# Autodesk Inventor assembly: Lever
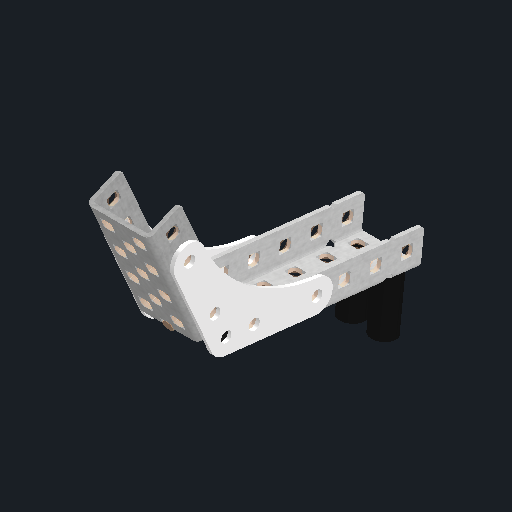
[picture p0: Inventor's stored thumbnail of the model, 512x512]
Saved by Autodesk Inventor 2025 (Build 290162000, 162)
## iProperties
Created: 2024-10-22
Part Number: Lever
Document SubType Name: Assembly
Designer: averey
Author: averey
## Documents named in this file (9)
- D:\VEX\High Stakes\CAD\V2\Clamp\Lever.iam
- D:\VEX\High Stakes\CAD\ROBOPROS-CAD-Inventor\Structure\C Channel\Aluminum 1x2x1\Alu C 1x2x1x5.ipt
- D:\VEX\High Stakes\CAD\V2\Clamp\Custom Parts\60 Degree Gusset.ipt
- D:\VEX\High Stakes\CAD\ROBOPROS-CAD-Inventor\Structure\Standoff\Standoff 1.00.ipt
- C:\Users\avere\VEX\High Stakes\CAD\ROBOPROS-CAD-Inventor\Structure\Standoff.ipt
- D:\VEX\High Stakes\CAD\ROBOPROS-CAD-Inventor\Structure\C Channel\Aluminum 1x2x1\Alu C 1x2x1x4.ipt
- D:\VEX\High Stakes\CAD\ROBOPROS-CAD-Inventor\Structure\C Channel\Aluminum 1x2x1\Alu C 1x2x1x6.ipt
- D:\VEX\High Stakes\CAD\ROBOPROS-CAD-Inventor\Motion\Spacers\Spacer Nylon .375 OD.ipt
- D:\VEX\High Stakes\CAD\ROBOPROS-CAD-Inventor\Motion\Spacers\Spacer Nylon .375 OD\NSpacer .375 OD x .875.ipt
## Components (8 placed, 6 different names)
1. Alu C 1x2x1x5:2 — Insert:2, Mate:1, Insert:3, Mate:3, Insert:6, Mate:7
2. 60 Degree Gusset:1 — Insert:2, Mate:1, Mate:5, Insert:5, Mate:6
3. 60 Degree Gusset:2 — Insert:3, Mate:3, Insert:4
4. Standoff 1.00:1 — Insert:4, Mate:5
5. Alu C 1x2x1x4:1 — Insert:5, Mate:6
6. Alu C 1x2x1x6:1 — Insert:6, Mate:7, Insert:7, Insert:8
7. NSpacer .375 OD x .875:1 — Insert:7
8. NSpacer .375 OD x .875:2 — Insert:8
## Relationships (12: Insert 7, Mate 5)
- Insert:2: Alu C 1x2x1x5:2 ↔ 60 Degree Gusset:1
- Mate:1: Alu C 1x2x1x5:2 ↔ 60 Degree Gusset:1
- Insert:3: Alu C 1x2x1x5:2 ↔ 60 Degree Gusset:2
- Mate:3: Alu C 1x2x1x5:2 ↔ 60 Degree Gusset:2
- Insert:4: 60 Degree Gusset:2 ↔ Standoff 1.00:1
- Mate:5: 60 Degree Gusset:1 ↔ Standoff 1.00:1
- Insert:5: 60 Degree Gusset:1 ↔ Alu C 1x2x1x4:1
- Mate:6: 60 Degree Gusset:1 ↔ Alu C 1x2x1x4:1
- Insert:6: Alu C 1x2x1x5:2 ↔ Alu C 1x2x1x6:1
- Mate:7: Alu C 1x2x1x5:2 ↔ Alu C 1x2x1x6:1
- Insert:7: Alu C 1x2x1x6:1 ↔ NSpacer .375 OD x .875:1
- Insert:8: Alu C 1x2x1x6:1 ↔ NSpacer .375 OD x .875:2
